# Autodesk Inventor assembly: SubAssembly - EntireLandingSystem
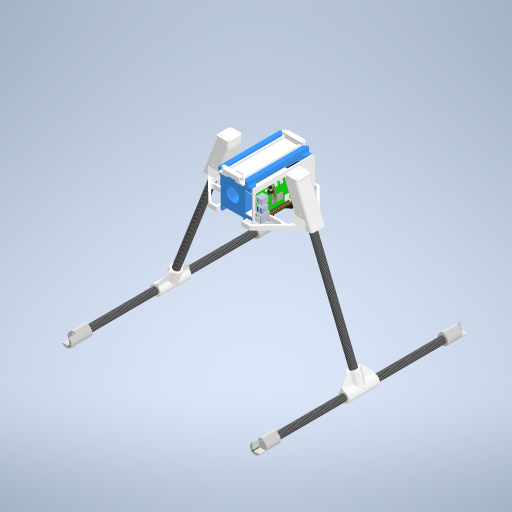
[picture p0: Inventor's stored thumbnail of the model, 512x512]
Saved by Autodesk Inventor 2023 (Build 270158000, 158)
## iProperties
Created: 2023-01-22
Part Number: SubAssembly - EntireLandingSystem
Document SubType Name: Assembly
Designer: Administrator
Author: Administrator
## Documents named in this file (6)
- C:\Users\chase\OneDrive\Documents\GitHub\WU-Team20-AutonomousDrone\CAD\ASSEMBLY\SubAssembly - EntireLandingSystem.iam
- C:\Users\chase\OneDrive\Documents\GitHub\WU-Team20-AutonomousDrone\CAD\ASSEMBLY\SubAssembly - Leg SingleSide.iam
- C:\Users\chase\OneDrive\Documents\GitHub\WU-Team20-AutonomousDrone\CAD\ASSEMBLY\SubAssembly - BatteryCarrier WithAccessories.iam
- C:\Users\chase\OneDrive\Documents\GitHub\WU-Team20-AutonomousDrone\CAD\Raw Models\AntiVibrationMount.ipt
- C:\Users\chase\OneDrive\Documents\GitHub\WU-Team20-AutonomousDrone\CAD\Legs\Foot1Assembly.iam
- C:\Users\chase\OneDrive\Documents\GitHub\WU-Team20-AutonomousDrone\CAD\Legs\Foot2Assembly.iam
## Components (8 placed, 5 different names)
1. SubAssembly - Leg SingleSide:1 [sub-assembly] — Rigid:2, Insert:2, Insert:3
2. SubAssembly - Leg SingleSide:2 [sub-assembly] — Rigid:3, Insert:1, Insert:4
3. SubAssembly - BatteryCarrier WithAccessories:1 [sub-assembly] — Rigid:2, Rigid:3, Rigid:4
4. AntiVibrationMount:1 — Rigid:4
5. Foot1Assembly:1 [sub-assembly] — Insert:1
6. Foot1Assembly:2 [sub-assembly] — Insert:2
7. Foot2Assembly:1 [sub-assembly] — Insert:3
8. Foot2Assembly:2 [sub-assembly] — Insert:4
## Relationships (7: Insert 4, WeldJoint 3)
- Rigid:2 [WeldJoint]: SubAssembly - Leg SingleSide:1 ↔ SubAssembly - BatteryCarrier WithAccessories:1
- Rigid:3 [WeldJoint]: SubAssembly - Leg SingleSide:2 ↔ SubAssembly - BatteryCarrier WithAccessories:1
- Rigid:4 [WeldJoint] (-5 mm): SubAssembly - BatteryCarrier WithAccessories:1 ↔ AntiVibrationMount:1
- Insert:1: SubAssembly - Leg SingleSide:2 ↔ Foot1Assembly:1
- Insert:2: SubAssembly - Leg SingleSide:1 ↔ Foot1Assembly:2
- Insert:3: SubAssembly - Leg SingleSide:1 ↔ Foot2Assembly:1
- Insert:4: SubAssembly - Leg SingleSide:2 ↔ Foot2Assembly:2
